# Autodesk Inventor assembly: dynamixel_pro_frame
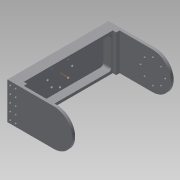
[picture p0: Inventor's stored thumbnail of the model, 180x180]
Saved by Autodesk Inventor 2017 (Build 210142000, 142)
## iProperties
Part Number: dynamixel_pro_frame
Material: Generisch
Document SubType Name: Assembly
Designer: Max
Author: Max
## Documents named in this file (4)
- C:\Users\Max\Desktop\SENAI\robot_arm_new\dynamixel_pro_frame.iam
- C:\Users\Max\Desktop\SENAI\robot_arm_new\dynamixel_pro_frame_part1.ipt
- C:\Users\Max\Desktop\SENAI\robot_arm_new\dynamixel_pro_frame_part2.ipt
- C:\Users\Max\Desktop\SENAI\robot_arm_new\dynamixel_pro_frame_part3.ipt
## Components (3 placed, 3 different names)
1. dynamixel_pro_frame_part1:1 — Passend:1, Passend:2, Passend:3, Passend:4, Passend:5, Passend:6, Passend:7, Passend:8, Passend:9
2. dynamixel_pro_frame_part2:1 — Passend:1, Passend:2, Passend:3
3. dynamixel_pro_frame_part3:1 — Passend:4, Passend:5, Passend:6
## Relationships (9: Mate 9)
- Passend:1 [Mate]: dynamixel_pro_frame_part1:1 ↔ dynamixel_pro_frame_part2:1
- Passend:2 [Mate]: dynamixel_pro_frame_part1:1 ↔ dynamixel_pro_frame_part2:1
- Passend:3 [Mate]: dynamixel_pro_frame_part1:1 ↔ dynamixel_pro_frame_part2:1
- Passend:4 [Mate]: dynamixel_pro_frame_part1:1 ↔ dynamixel_pro_frame_part3:1
- Passend:5 [Mate]: dynamixel_pro_frame_part1:1 ↔ dynamixel_pro_frame_part3:1
- Passend:6 [Mate]: dynamixel_pro_frame_part1:1 ↔ dynamixel_pro_frame_part3:1
- Passend:7 [Mate]: dynamixel_pro_frame_part1:1
- Passend:8 [Mate]: dynamixel_pro_frame_part1:1
- Passend:9 [Mate]: dynamixel_pro_frame_part1:1
